# Autodesk Inventor assembly: Montagem quase pronto
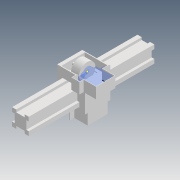
[picture p0: Inventor's stored thumbnail of the model, 180x180]
Saved by Autodesk Inventor 2021 (Build 250183000, 183)
## iProperties
Created: 2020-10-21
Part Number: Montagem quase pronto
Document SubType Name: Assembly
Designer: evert
Author: evert
## Documents named in this file (5)
- C:\Users\evert\OneDrive\Área de Trabalho\peca move\Montagem quase pronto.iam
- C:\Users\evert\OneDrive\Área de Trabalho\peca move\Peça16.ipt
- C:\Users\evert\OneDrive\Área de Trabalho\peca move\roda certa.ipt
- C:\Users\evert\OneDrive\Área de Trabalho\peca move\Viga_Projeto_Bosch.ipt
- C:\Users\evert\OneDrive\Área de Trabalho\peca move\Servo Motor SG90.ipt
## Components (4 placed, 4 different names)
1. Peça16:1 — Rotativa:1
2. Viga_Projeto_Bosch:1
3. roda certa:1 — Rotativa:1
4. Servo Motor SG90:1
## Relationships (1: RevoluteJoint 1)
- Rotativa:1 [RevoluteJoint]: Peça16:1 ↔ roda certa:1
